# Autodesk Inventor assembly: Z25_Folding_Arm
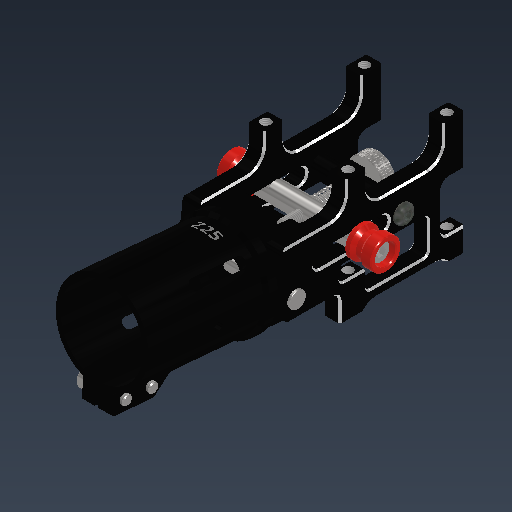
[picture p0: Inventor's stored thumbnail of the model, 512x512]
Saved by Autodesk Inventor 2024.1 (Build 281209000, 209)
## iProperties
Created: 2023-12-11
Part Number: Z25_Folding_Arm
Document SubType Name: Assembly
Designer: dzw04
Mass: 75.035 g
Surface Area: 230.57 cm^2
Volume: 23.1949 cm^3
Density: 3.23497 g/cm^3
Author: dzw04
## Documents named in this file (15)
- C:\Users\dzw04\Saxion\Mechatronica Lectoraat LMECH LED - Database ARG\Component_Database\SARAX\01. CAD\01. 3D_Drawing\02. Sub_Assemblies\Z25_Folding_Arm\Z25_Folding_Arm.iam
- C:\Users\dzw04\Saxion\Mechatronica Lectoraat LMECH LED - Database ARG\Component_Database\SARAX\01. CAD\01. 3D_Drawing\02. Sub_Assemblies\Z25_Folding_Arm\01. Parts\Z25_Sideplate.ipt
- C:\Users\dzw04\Saxion\Mechatronica Lectoraat LMECH LED - Database ARG\Component_Database\SARAX\01. CAD\01. 3D_Drawing\02. Sub_Assemblies\Z25_Folding_Arm\01. Parts\Z25_Pipe_Clamp.ipt
- C:\Users\dzw04\Saxion\Mechatronica Lectoraat LMECH LED - Database ARG\Component_Database\SARAX\01. CAD\01. 3D_Drawing\02. Sub_Assemblies\Z25_Folding_Arm\01. Parts\Z25_Hinge_Shaft.ipt
- C:\Users\dzw04\Saxion\Mechatronica Lectoraat LMECH LED - Database ARG\Component_Database\SARAX\01. CAD\01. 3D_Drawing\02. Sub_Assemblies\Z25_Folding_Arm\01. Parts\Z25_Side_Lock_Button.ipt
- C:\Users\dzw04\Saxion\Mechatronica Lectoraat LMECH LED - Database ARG\Component_Database\SARAX\01. CAD\01. 3D_Drawing\02. Sub_Assemblies\Z25_Folding_Arm\01. Parts\Z25_Slide_Shaft.ipt
- C:\Users\dzw04\Saxion\Mechatronica Lectoraat LMECH LED - Database ARG\Component_Database\SARAX\01. CAD\01. 3D_Drawing\02. Sub_Assemblies\Z25_Folding_Arm\01. Parts\Z25_Slide_Spacer.ipt
- C:\Users\dzw04\Saxion\Mechatronica Lectoraat LMECH LED - Database ARG\Component_Database\SARAX\01. CAD\01. 3D_Drawing\02. Sub_Assemblies\Z25_Folding_Arm\01. Parts\Z25_Spacer.ipt
- C:\Users\dzw04\Saxion\Mechatronica Lectoraat LMECH LED - Database ARG\Component_Database\SARAX\01. CAD\01. 3D_Drawing\01. Parts\en-US\ISO 4762(2)\ISO 4762 - M3 x 8ISO.ipt
- C:\Users\dzw04\Saxion\Mechatronica Lectoraat LMECH LED - Database ARG\Component_Database\SARAX\01. CAD\01. 3D_Drawing\01. Parts\en-US\BS 4464 B\BS 4464 - M2,5 Form B.ipt
- C:\Users\dzw04\Saxion\Mechatronica Lectoraat LMECH LED - Database ARG\Component_Database\SARAX\01. CAD\01. 3D_Drawing\01. Parts\en-US\ISO 7045  H\ISO 7045 - M2,5 x 5_ - 4.8 - H - ISO.ipt
- C:\Users\dzw04\Saxion\Mechatronica Lectoraat LMECH LED - Database ARG\Component_Database\SARAX\01. CAD\01. 3D_Drawing\01. Parts\en-US\ISO 7380-1\ISO 7380-1 - M3 x 6.ipt
- C:\Users\dzw04\Saxion\Mechatronica Lectoraat LMECH LED - Database ARG\Component_Database\SARAX\01. CAD\01. 3D_Drawing\01. Parts\en-US\ISO 4762(2)\ISO 4762 - M3 x 10ISO.ipt
- C:\Users\dzw04\Saxion\Mechatronica Lectoraat LMECH LED - Database ARG\Component_Database\SARAX\01. CAD\01. 3D_Drawing\02. Sub_Assemblies\Z25_Folding_Arm\01. Parts\Z25_Spring.ipt
- C:\Users\dzw04\Saxion\Mechatronica Lectoraat LMECH LED - Database ARG\Component_Database\SARAX\01. CAD\01. 3D_Drawing\Parameters.xlsx
## Components (18 placed, 13 different names)
1. Z25_Sideplate:1 — Mate:1, Flush:1, Flush:2, Mate:6, Flush:3, Angle:2, Mate:13, Mate:14, Insert:5
2. Z25_Sideplate:2 — Mate:1, Flush:1, Flush:2, Mate:2, Mate:3, Angle:1, Mate:4, Mate:5, Insert:4
3. Z25_Pipe_Clamp:1 — Mate:2, Mate:3, Angle:1, Insert:6, Insert:7
4. Z25_Hinge_Shaft:1 — Mate:13, Mate:14, Mate:15, Mate:16
5. Z25_Side_Lock_Button:1 — Mate:9, Mate:12, Insert:1
6. Z25_Side_Lock_Button:2 — Mate:10, Mate:11, Insert:2
7. Z25_Slide_Shaft:1 — Flush:4, Mate:7, Mate:17
8. Z25_Slide_Spacer:1 — Mate:6, Flush:3, Mate:8, Mate:9, Mate:10, Mate:11, Mate:12
9. Z25_Spacer:1 — Mate:4, Mate:5, Angle:2, Flush:4, Mate:7, Mate:8, Flush:5
10. ISO 4762 M3 x 8:1 — Insert:1
11. ISO 4762 M3 x 8:2 — Insert:2
12. BS 4464 Form B M2,5 Form B:1 — Mate:15, Mate:16, Insert:3
13. ISO 7045 H M2,5 x 5 - 4.8 - H:1 — Insert:3
14. ISO 7380-1 M3 x 6:1 — Insert:4
15. ISO 7380-1 M3 x 6:2 — Insert:5
16. ISO 4762 M3 x 10:1 — Insert:6
17. ISO 4762 M3 x 10:2 — Insert:7
18. Z25_Spring:1 — Mate:17, Flush:5
## Relationships (31: Mate 17, Insert 7, Flush 5, Angle 2)
- Mate:1 (20 mm): Z25_Sideplate:1 ↔ Z25_Sideplate:2
- Flush:1: Z25_Sideplate:1 ↔ Z25_Sideplate:2
- Flush:2: Z25_Sideplate:1 ↔ Z25_Sideplate:2
- Mate:2: Z25_Sideplate:2 ↔ Z25_Pipe_Clamp:1
- Mate:3: Z25_Sideplate:2 ↔ Z25_Pipe_Clamp:1
- Angle:1 (5 deg): Z25_Sideplate:2 ↔ Z25_Pipe_Clamp:1
- Mate:4: Z25_Sideplate:2 ↔ Z25_Spacer:1
- Mate:5: Z25_Sideplate:2 ↔ Z25_Spacer:1
- Mate:6 (0.25 mm): Z25_Sideplate:1 ↔ Z25_Slide_Spacer:1
- Flush:3 (-0.5 mm): Z25_Sideplate:1 ↔ Z25_Slide_Spacer:1
- Angle:2 (0 deg): Z25_Sideplate:1 ↔ Z25_Spacer:1
- Flush:4 (5 mm): Z25_Slide_Shaft:1 ↔ Z25_Spacer:1
- Mate:7: Z25_Slide_Shaft:1 ↔ Z25_Spacer:1
- Mate:8 (10 mm): Z25_Slide_Spacer:1 ↔ Z25_Spacer:1
- Mate:9: Z25_Side_Lock_Button:1 ↔ Z25_Slide_Spacer:1
- Mate:10: Z25_Side_Lock_Button:2 ↔ Z25_Slide_Spacer:1
- Mate:11: Z25_Side_Lock_Button:2 ↔ Z25_Slide_Spacer:1
- Mate:12: Z25_Side_Lock_Button:1 ↔ Z25_Slide_Spacer:1
- Mate:13: Z25_Sideplate:1 ↔ Z25_Hinge_Shaft:1
- Mate:14: Z25_Sideplate:1 ↔ Z25_Hinge_Shaft:1
- Insert:1: Z25_Side_Lock_Button:1 ↔ ISO 4762 M3 x 8:1
- Insert:2: Z25_Side_Lock_Button:2 ↔ ISO 4762 M3 x 8:2
- Mate:15: Z25_Hinge_Shaft:1 ↔ BS 4464 Form B M2,5 Form B:1
- Mate:16: Z25_Hinge_Shaft:1 ↔ BS 4464 Form B M2,5 Form B:1
- Insert:3: BS 4464 Form B M2,5 Form B:1 ↔ ISO 7045 H M2,5 x 5 - 4.8 - H:1
- Insert:4: Z25_Sideplate:2 ↔ ISO 7380-1 M3 x 6:1
- Insert:5: Z25_Sideplate:1 ↔ ISO 7380-1 M3 x 6:2
- Insert:6: Z25_Pipe_Clamp:1 ↔ ISO 4762 M3 x 10:1
- Insert:7: Z25_Pipe_Clamp:1 ↔ ISO 4762 M3 x 10:2
- Mate:17: Z25_Slide_Shaft:1 ↔ Z25_Spring:1
- Flush:5 (0.25 mm): Z25_Spacer:1 ↔ Z25_Spring:1
## Named parameters: BatteryLength = 200 mm, BatteryWidth = 62 mm, BatteryHeight = 76 mm, NumberOfArms = 4, RotorToRotor = 900 mm, MountToMotorCenter = 0 mm, ArmPosition = 5 deg, ThicknessBodyCenterPlate = 2 mm, ThicknessBodyOuterPlate = 2 mm, ThicknessLegLoadpipePlate = 2 mm, ThicknessBatteryTray = 2 mm, ThicknessBatteryTopTray = 1 mm, LoadpipeLength = 450 mm, NumberOfBatterys = 2, LandingGearStabilityBar = 525 mm, LandingGearRod = 390 mm, LandingGearHeight = 400 mm, StartAngleArm = 45 deg, MotorMountCenter = 71.5 mm
